# Autodesk Inventor assembly: Assembly3
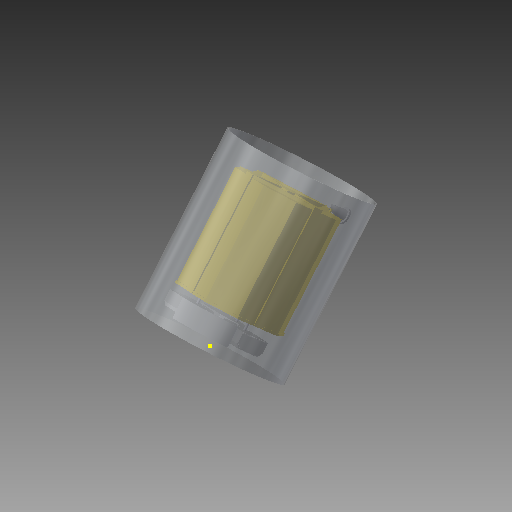
[picture p0: Inventor's stored thumbnail of the model, 512x512]
Saved by Autodesk Inventor 2018 (Build 220112000, 112)
## iProperties
Created: 2021-03-16
Part Number: Assembly3
Document SubType Name: Assembly
Designer: dell
Author: dell
## Documents named in this file (3)
- D:\Autodesk\Projects\C-C\a1\ES101 GROUP-13 PROJECT\FINAL MODEL\Resolved files\Assembly3.iam
- D:\Autodesk\Projects\C-C\a1\ES101 GROUP-13 PROJECT\FINAL MODEL\Resolved files\Assembly2.iam
- D:\Autodesk\Projects\C-C\a1\ES101 GROUP-13 PROJECT\INDIVIDUAL WORK\Tejas\Resolved files\Derived Middle TC.ipt
## Components (2 placed, 2 different names)
1. Assembly2:1 [sub-assembly] — Mate:1
2. Derived Middle TC:1 — Mate:1
## Relationships (1: Mate 1)
- Mate:1 (2 mm): Assembly2:1 ↔ Derived Middle TC:1
